# Autodesk Inventor assembly: bearing mount on extrsusion
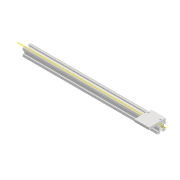
[picture p0: Inventor's stored thumbnail of the model, 180x180]
Saved by Autodesk Inventor 2020 (Build 240168000, 168)
## iProperties
Created: 2019-12-20
Part Number: bearing mount on extrsusion
Document SubType Name: Assembly
Designer: ball
Author: ball
## Documents named in this file (4)
- C:\FTC\FTC8863CAD\2019 Robot\Collection\bearing mount on extrsusion.iam
- C:\FTC\FTC8863CAD\Actobotics\565 parts\565046.ipt
- C:\FTC\FTC8863CAD\2019 Robot\Collection\Bearing mount for xrail.ipt
- C:\FTC\FTC8863CAD\Actobotics\585 parts\585757.ipt
## Components (3 placed, 3 different names)
1. 565046:1 — Flush:1, Flush:2, Flush:3, Mate:1, Flush:4
2. Bearing mount for xrail:1 — Flush:1, Flush:2
3. 585757:1 — Flush:3, Mate:1, Flush:4
## Relationships (5: Flush 4, Mate 1)
- Flush:1: 565046:1 ↔ Bearing mount for xrail:1
- Flush:2: 565046:1 ↔ Bearing mount for xrail:1
- Flush:3: 565046:1 ↔ 585757:1
- Mate:1: 565046:1 ↔ 585757:1
- Flush:4: 565046:1 ↔ 585757:1
